# Autodesk Inventor assembly: TruckMotorWheelEtc
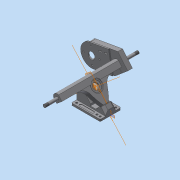
[picture p0: Inventor's stored thumbnail of the model, 180x180]
Saved by Autodesk Inventor 2017 (Build 210142000, 142)
## iProperties
Created: 2016-12-25
Part Number: TruckMotorWheelEtc
Document SubType Name: Assembly
Designer: Joshua Yuan
Author: Joshua Yuan
## Documents named in this file (4)
- C:\Other Project Stuff\Longboard\TruckMotorWheelEtc.iam
- C:\Other Project Stuff\Longboard\MMplates.iam
- C:\Other Project Stuff\Longboard\50cal_truck.ipt
- C:\Other Project Stuff\Longboard\50cal_baseplate.ipt
## Components (3 placed, 3 different names)
1. MMplates:1 [sub-assembly] — Mate:4, Mate:5
2. 50cal_truck:1 — Mate:2, Mate:3, Mate:4, Mate:5
3. 50cal_baseplate:1 — Mate:2, Mate:3
## Relationships (4: Mate 4)
- Mate:2: 50cal_truck:1 ↔ 50cal_baseplate:1
- Mate:3: 50cal_truck:1 ↔ 50cal_baseplate:1
- Mate:4: MMplates:1 ↔ 50cal_truck:1
- Mate:5: MMplates:1 ↔ 50cal_truck:1
